# Autodesk Inventor assembly: Assembly_RWACS
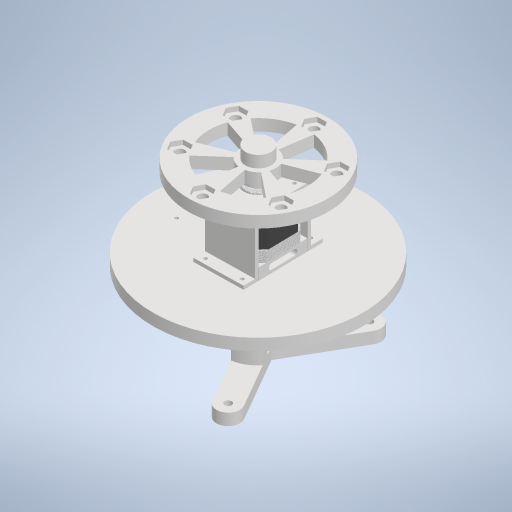
[picture p0: Inventor's stored thumbnail of the model, 512x512]
Saved by Autodesk Inventor 2023 (Build 270158000, 158)
## iProperties
Created: 2022-12-10
Part Number: Assembly_RWACS
Document SubType Name: Assembly
Designer: Krzysztof
Author: Krzysztof
## Documents named in this file (7)
- C:\Users\Krzysztof\Documents\RWACS_invertor\Assembly_RWACS.iam
- C:\Users\Krzysztof\Documents\RWACS_invertor\Base.ipt
- C:\Users\Krzysztof\Documents\RWACS_invertor\Motor_cage.ipt
- C:\Users\Krzysztof\Documents\RWACS_invertor\Reaction_wheel.ipt
- C:\Users\Krzysztof\Documents\RWACS_invertor\Satellite_plate.ipt
- C:\Users\Krzysztof\Documents\Inventor\Content Center Files\R2023\en-US\DIN 615\DIN 615 - L 25 - 25 x 52 x 15.ipt
- C:\Users\Krzysztof\Documents\RWACS_invertor\stepper-motor-nema17-17hs4401-42-mm-1.snapshot.1\Assembly1.iam
## Components (6 placed, 6 different names)
1. Base:1 — Mate:1, Mate:2, Mate:3, Insert:1
2. Motor_cage:1 — Mate:5, Flush:3, Mate:7
3. Reaction_wheel:1 — Insert:3
4. Satellite_plate:1 — Insert:2, Flush:1, Flush:2, Mate:5, Flush:3, Mate:6, Mate:7
5. DIN 615 L 25 - 25 x 52 x 15:1 — Insert:1, Insert:2
6. Assembly1:1 [sub-assembly] — Flush:1, Flush:2, Insert:3, Mate:6
## Relationships (12: Mate 6, Insert 3, Flush 3)
- Mate:1: Base:1
- Mate:2: Base:1
- Mate:3: Base:1
- Insert:1: Base:1 ↔ DIN 615 L 25 - 25 x 52 x 15:1
- Insert:2: Satellite_plate:1 ↔ DIN 615 L 25 - 25 x 52 x 15:1
- Flush:1: Satellite_plate:1 ↔ Assembly1:1
- Flush:2: Satellite_plate:1 ↔ Assembly1:1
- Mate:5 (0.35 mm): Motor_cage:1 ↔ Satellite_plate:1
- Flush:3: Motor_cage:1 ↔ Satellite_plate:1
- Insert:3: Reaction_wheel:1 ↔ Assembly1:1
- Mate:6: Satellite_plate:1 ↔ Assembly1:1
- Mate:7: Motor_cage:1 ↔ Satellite_plate:1
